# Autodesk Inventor assembly: Maccaronikanone
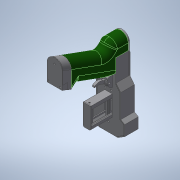
[picture p0: Inventor's stored thumbnail of the model, 180x180]
Saved by Autodesk Inventor 2021 (Build 250183000, 183)
## iProperties
Created: 2021-03-07
Part Number: Maccaronikanone
Document SubType Name: Assembly
Designer: Lukas
Author: Lukas
## Documents named in this file (21)
- Z:\Datastorrage\Projects\Maccaroni-Gun\Inventor files\Maccaronikanone.iam
- Z:\Datastorrage\Projects\Maccaroni-Gun\Inventor files\Maccaroni.ipt
- Z:\Datastorrage\Projects\Maccaroni-Gun\Inventor files\Motor_18mm.ipt
- Z:\Datastorrage\Projects\Maccaroni-Gun\Inventor files\Motor_holder.ipt
- Z:\Datastorrage\Projects\Maccaroni-Gun\Inventor files\Antriebsrad.ipt
- Z:\Datastorrage\Projects\Maccaroni-Gun\Inventor files\Abzugsgehäuse.ipt
- Z:\Datastorrage\Projects\Maccaroni-Gun\Inventor files\Magazin.ipt
- Z:\Datastorrage\Projects\Maccaroni-Gun\Inventor files\Magazin_Stössel.ipt
- Z:\Datastorrage\Projects\Maccaroni-Gun\Inventor files\Magazin_Boden.ipt
- Z:\Datastorrage\Projects\Maccaroni-Gun\Inventor files\Griff.ipt
- Z:\Datastorrage\Projects\Maccaroni-Gun\Inventor files\Hammer_Halter.ipt
- Z:\Datastorrage\Projects\Maccaroni-Gun\Inventor files\Abzug2.ipt
- Z:\Datastorrage\Projects\Maccaroni-Gun\Inventor files\Hammer2.ipt
- Z:\Datastorrage\Projects\Maccaroni-Gun\Inventor files\Abzughalter.ipt
- Z:\Datastorrage\Projects\Maccaroni-Gun\Inventor files\Top_Lid.ipt
- Z:\Datastorrage\Projects\Maccaroni-Gun\Inventor files\Stiftleiste_3Pin.ipt
- Z:\Datastorrage\Projects\Maccaroni-Gun\Inventor files\Stiftleiste_Halter.ipt
- Z:\Datastorrage\Projects\Maccaroni-Gun\Inventor files\ESC_Halter.ipt
- Z:\Datastorrage\Projects\Maccaroni-Gun\Inventor files\Arduinohalter.ipt
- Z:\Datastorrage\Projects\Maccaroni-Gun\Inventor files\Hauptschalter.ipt
- Z:\Datastorrage\Projects\Maccaroni-Gun\Inventor files\Ladesteckerhalter.ipt
## Components (24 placed, 20 different names)
1. Abzugsgehäuse:1 — Flush:1, Flush:2, Flush:3, Mate:61, Mate:62, Angle:1, Angle:2, Mate:69, Mate:70, Flush:6, Mate:72, Mate:76, Mate:82, Mate:83, Mate:84, Mate:86, Mate:88, Mate:89, Mate:90, Flush:10, Mate:93, Mate:94, Mate:96, Mate:98, Mate:99, Flush:11, Flush:12, Mate:102, Mate:103, Flush:13, Flush:14, Mate:104, Mate:105, Mate:108, Mate:109
2. Maccaroni:1 — Mate:63, Mate:70, Mate:71
3. Motor_holder:1 — Mate:55, Mate:56, Mate:57, Mate:58, Mate:59, Mate:60, Mate:61, Mate:62, Angle:1
4. Motor_18mm:1 — Mate:58, Mate:59, Mate:60, Insert:2, Mate:64
5. Motor_18mm:2 — Mate:55, Mate:56, Mate:57, Insert:1, Mate:65
6. Antriebsrad:1 — Insert:1, Mate:65
7. Antriebsrad:2 — Insert:2, Mate:64
8. Magazin:1 — Angle:2, Mate:68, Mate:95, Mate:69, Mate:71, Flush:6, Mate:72, Flush:7, Mate:73, Flush:8, Mate:96, Mate:97
9. Magazin_Stössel:1 — Mate:68, Mate:95, Mate:97
10. Magazin_Boden:1 — Flush:7, Mate:73, Flush:8
11. Griff:1 — Mate:76, Mate:91, Mate:92, Mate:93, Mate:94, Mate:117, Mate:118
12. Hammer_Halter:1 — Mate:82, Mate:83, Mate:84, Mate:87, Angle:3
13. Abzug2:1 — Mate:85, Mate:86, Tangent:1
14. Hammer2:1 — Mate:87, Angle:3, Tangent:1
15. Abzughalter:1 — Mate:88, Mate:85, Mate:89, Mate:90
16. Top_Lid:1 — Mate:91, Flush:10, Mate:92, Mate:107, Mate:112, Mate:113, Mate:114
17. Stiftleiste_Halter:1 — Mate:103, Flush:13, Mate:105, Mate:106
18. Stiftleiste_Halter:2 — Mate:102, Flush:14, Mate:104, Flush:15
19. Stiftleiste_3Pin:1 — Mate:99, Flush:11, Mate:106
20. Stiftleiste_3Pin:2 — Mate:98, Flush:12, Flush:15
21. ESC_Halter:1 — Mate:107, Mate:108, Mate:109
22. Arduinohalter:1 — Mate:112, Mate:113, Mate:114
23. Hauptschalter:1 — Mate:117, Mate:118, Mate:119, Mate:120, Mate:121
24. Ladesteckerhalter:1 — Mate:119, Mate:120, Mate:121
## Relationships (70: Mate 52, Flush 12, Angle 3, Insert 2, Tangent 1)
- Flush:1: Abzugsgehäuse:1
- Flush:2: Abzugsgehäuse:1
- Flush:3: Abzugsgehäuse:1
- Mate:55: Motor_holder:1 ↔ Motor_18mm:2
- Mate:56: Motor_holder:1 ↔ Motor_18mm:2
- Mate:57: Motor_holder:1 ↔ Motor_18mm:2
- Mate:58: Motor_holder:1 ↔ Motor_18mm:1
- Mate:59: Motor_holder:1 ↔ Motor_18mm:1
- Mate:60: Motor_holder:1 ↔ Motor_18mm:1
- Mate:61: Abzugsgehäuse:1 ↔ Motor_holder:1
- Mate:62: Abzugsgehäuse:1 ↔ Motor_holder:1
- Angle:1 (0 deg): Abzugsgehäuse:1 ↔ Motor_holder:1
- Mate:63: Maccaroni:1
- Insert:1: Motor_18mm:2 ↔ Antriebsrad:1
- Insert:2: Motor_18mm:1 ↔ Antriebsrad:2
- Mate:64: Motor_18mm:1 ↔ Antriebsrad:2
- Mate:65: Motor_18mm:2 ↔ Antriebsrad:1
- Angle:2 (180 deg): Abzugsgehäuse:1 ↔ Magazin:1
- Mate:68: Magazin:1 ↔ Magazin_Stössel:1
- Mate:95: Magazin:1 ↔ Magazin_Stössel:1
- Mate:69 (0.1 mm): Abzugsgehäuse:1 ↔ Magazin:1
- Mate:70 (13 mm): Abzugsgehäuse:1 ↔ Maccaroni:1
- Mate:71: Maccaroni:1 ↔ Magazin:1
- Flush:6: Abzugsgehäuse:1 ↔ Magazin:1
- Mate:72: Abzugsgehäuse:1 ↔ Magazin:1
- Flush:7: Magazin:1 ↔ Magazin_Boden:1
- Mate:73: Magazin:1 ↔ Magazin_Boden:1
- Flush:8: Magazin:1 ↔ Magazin_Boden:1
- Mate:76: Abzugsgehäuse:1 ↔ Griff:1
- Mate:82: Abzugsgehäuse:1 ↔ Hammer_Halter:1
- Mate:83: Abzugsgehäuse:1 ↔ Hammer_Halter:1
- Mate:84: Abzugsgehäuse:1 ↔ Hammer_Halter:1
- Mate:85: Abzug2:1 ↔ Abzughalter:1
- Mate:86 (0.1 mm): Abzugsgehäuse:1 ↔ Abzug2:1
- Mate:87: Hammer_Halter:1 ↔ Hammer2:1
- Angle:3 (0 deg): Hammer_Halter:1 ↔ Hammer2:1
- Tangent:1: Abzug2:1 ↔ Hammer2:1
- Mate:88: Abzugsgehäuse:1 ↔ Abzughalter:1
- Mate:89: Abzugsgehäuse:1 ↔ Abzughalter:1
- Mate:90: Abzugsgehäuse:1 ↔ Abzughalter:1
- Mate:91 (0.2 mm): Griff:1 ↔ Top_Lid:1
- Flush:10: Abzugsgehäuse:1 ↔ Top_Lid:1
- Mate:92: Griff:1 ↔ Top_Lid:1
- Mate:93: Abzugsgehäuse:1 ↔ Griff:1
- Mate:94: Abzugsgehäuse:1 ↔ Griff:1
- Mate:96: Abzugsgehäuse:1 ↔ Magazin:1
- Mate:97: Magazin:1 ↔ Magazin_Stössel:1
- Mate:98: Abzugsgehäuse:1 ↔ Stiftleiste_3Pin:2
- Mate:99: Abzugsgehäuse:1 ↔ Stiftleiste_3Pin:1
- Flush:11: Abzugsgehäuse:1 ↔ Stiftleiste_3Pin:1
- Flush:12: Abzugsgehäuse:1 ↔ Stiftleiste_3Pin:2
- Mate:102 (0.2 mm): Abzugsgehäuse:1 ↔ Stiftleiste_Halter:2
- Mate:103 (0.2 mm): Abzugsgehäuse:1 ↔ Stiftleiste_Halter:1
- Flush:13: Abzugsgehäuse:1 ↔ Stiftleiste_Halter:1
- Flush:14: Abzugsgehäuse:1 ↔ Stiftleiste_Halter:2
- Mate:104: Abzugsgehäuse:1 ↔ Stiftleiste_Halter:2
- Mate:105: Abzugsgehäuse:1 ↔ Stiftleiste_Halter:1
- Mate:106: Stiftleiste_Halter:1 ↔ Stiftleiste_3Pin:1
- Flush:15: Stiftleiste_Halter:2 ↔ Stiftleiste_3Pin:2
- Mate:107: Top_Lid:1 ↔ ESC_Halter:1
- Mate:108: Abzugsgehäuse:1 ↔ ESC_Halter:1
- Mate:109: Abzugsgehäuse:1 ↔ ESC_Halter:1
- Mate:112: Top_Lid:1 ↔ Arduinohalter:1
- Mate:113: Top_Lid:1 ↔ Arduinohalter:1
- Mate:114: Top_Lid:1 ↔ Arduinohalter:1
- Mate:117: Griff:1 ↔ Hauptschalter:1
- Mate:118: Griff:1 ↔ Hauptschalter:1
- Mate:119: Hauptschalter:1 ↔ Ladesteckerhalter:1
- Mate:120: Hauptschalter:1 ↔ Ladesteckerhalter:1
- Mate:121 (10.9 mm): Hauptschalter:1 ↔ Ladesteckerhalter:1
